# Autodesk Inventor assembly: Elo_sup
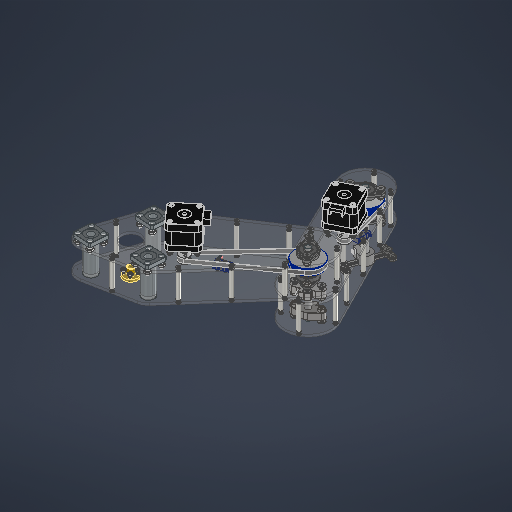
[picture p0: Inventor's stored thumbnail of the model, 512x512]
Saved by Autodesk Inventor 2025.2 (Build 292293000, 293)
## iProperties
Created: 2025-04-19
Part Number: Elo_sup
Document SubType Name: Assembly
Designer: Nelson
Author: Nelson
## Documents named in this file (33)
- C:\Users\Tiago\Documents\Inventor\Exp. Braço v1\Elo_sup.iam
- C:\Users\Tiago\Documents\Inventor\Exp. Braço v1\Veio_D8mm_L100mm.ipt
- C:\Users\Tiago\Documents\Inventor\Exp. Braço v1\RolamentoLinear10d.ipt
- C:\Users\Tiago\Documents\Inventor\Exp. Braço v1\KFL08 - Mancal Flange oval Ø8.ipt
- C:\Users\Tiago\Documents\Inventor\Exp. Braço v1\NEMA17 42-38.ipt
- C:\Users\Tiago\Documents\Inventor\Exp. Braço v1\Porca_T8.ipt
- C:\Users\Tiago\Documents\Inventor\Exp. Braço v1\Linear_Shaft_Support_SHF8.ipt
- C:\Users\Tiago\Documents\Inventor\Exp. Braço v1\1ELO.ipt
- C:\Users\Tiago\Documents\Inventor\Exp. Braço v1\2ELO.ipt
- C:\Users\Tiago\Documents\Inventor\Exp. Braço v1\3ELO.ipt
- C:\Users\Tiago\Documents\Inventor\Exp. Braço v1\4ELO.ipt
- C:\Users\Tiago\Documents\Inventor\Exp. Braço v1\espaçador_M3_L40.ipt
- C:\Users\Tiago\Documents\Inventor\Exp. Braço v1\GT2Pulley_z60.ipt
- C:\Users\Tiago\Documents\Inventor\Exp. Braço v1\GT2Pulley_z20.ipt
- C:\Users\Tiago\Documents\Inventor\Exp. Braço v1\Elo_sup\Design Accelerator\Synchronous Belts Transmission3.iam
- C:\Users\Tiago\Documents\Inventor\Exp. Braço v1\Elo_sup\Design Accelerator\Synchronous Belts Transmission5.iam
- C:\Users\Tiago\Documents\Inventor\Exp. Braço v1\M3 x0.5 ALT (...).ipt
- C:\Users\Tiago\Documents\Inventor\Exp. Braço v1\Anilha_M3.ipt
- C:\Users\Tiago\Documents\Inventor\Exp. Braço v1\M3 x8L_hexagonal_BigHEAD.ipt
- C:\Users\Tiago\Documents\Inventor\Exp. Braço v1\M5x14L_Hex.ipt
- C:\Users\Tiago\Documents\Inventor\Exp. Braço v1\M5_nylonLock_Nut.ipt
- C:\Users\Tiago\Documents\Inventor\Exp. Braço v1\M4x12L_Hex.ipt
- C:\Users\Tiago\Documents\Inventor\Exp. Braço v1\Porca_sextavada(4M).ipt
- C:\Users\Tiago\Documents\Inventor\Exp. Braço v1\M5x16L_Hex.ipt
- C:\Users\Tiago\Documents\Inventor\Exp. Braço v1\M2x12L_Hex.ipt
- M2x12L_Hex.ipt
- C:\Users\Tiago\Documents\Inventor\Exp. Braço v1\Porca_sextavada(M2).ipt
- C:\Users\Tiago\Documents\Inventor\Exp. Braço v1\M5 x12L_Hex_C.ipt
- M5 x12L_Hex_C.ipt
- C:\Users\Tiago\Documents\Inventor\Exp. Braço v1\Porca_sextavada(3M).ipt
- C:\Users\Tiago\Documents\Inventor\Exp. Braço v1\Limit switch\complete limit switch\complete limit switch\complete limit switch.ipt
- C:\Users\Tiago\Documents\Inventor\Exp. Braço v1\EndEffector_holder_Touch.ipt
- C:\Users\Tiago\Documents\Inventor\Exp. Braço v1\EndEffector_Holder_for_SHF.ipt
## Components (176 placed, 29 different names)
1. Veio_D8mm_L100mm:1 — Mate:45, Mate:48, Mate:61, Flush:3, Mate:64, Mate:65, Mate:78, Mate:82, Flush:5, Mate:143, Rotation:3, Rotation:4
2. RolamentoLinear10d:1 — Mate:54, Mate:68, Flush:4, Mate:192, Mate:193, Insert:163, Insert:168, Insert:169, Insert:170
3. RolamentoLinear10d:2 — Mate:56, Mate:190, Mate:191, Insert:159, Insert:160, Insert:161, Insert:162
4. RolamentoLinear10d:3 — Mate:57, Mate:70, Mate:194, Mate:195, Insert:164, Insert:165, Insert:166, Insert:167
5. KFL08 - Mancal Flange oval Ø8:1 — Mate:65, Mate:71, Mate:91, Insert:147, Insert:148
6. KFL08 - Mancal Flange oval Ø8:2 — Mate:63, Mate:64, Mate:74, Mate:75, Insert:149, Insert:150
7. NEMA17 42-38:1 — Mate:98, Mate:141, Mate:144, Flush:161, Mate:201, Mate:202, Mate:203, Mate:204
8. Porca_T8:1 — Mate:66, Mate:67, Mate:76, Mate:77, Insert:199, Insert:200, Insert:201, Insert:202
9. NEMA17 42-38:2 — Mate:162, Mate:163, Mate:164, Flush:159, Mate:197, Mate:198, Mate:199, Mate:200
10. Linear_Shaft_Support_SHF8:1 — Mate:45, Mate:80, Mate:81, Insert:187, Insert:188, Insert:195
11. Linear_Shaft_Support_SHF8:2 — Mate:48, Mate:83, Mate:84, Insert:189, Insert:190, Insert:196
12. Veio_D8mm_L100mm:2 — Mate:51, Mate:53, Mate:85, Mate:86, Flush:6, Mate:149, Flush:162, Mate:211
13. KFL08 - Mancal Flange oval Ø8:3 — Mate:51, Mate:87, Mate:88, Insert:157, Insert:158
14. KFL08 - Mancal Flange oval Ø8:4 — Mate:53, Mate:89, Mate:90, Insert:155, Insert:156
15. 1ELO:1 — Mate:54, Mate:56, Mate:57, Mate:61, Flush:3, Mate:63, Mate:74, Mate:75, Mate:98, Mate:100, Mate:101, Mate:102, Mate:103, Mate:104, Mate:105, Mate:106, Mate:121, Mate:127, Mate:144, Mate:145, Mate:146, Flush:158, Mate:157, Mate:186, Mate:187, Mate:188, Mate:189, Mate:190, Mate:191, Mate:192, Mate:193, Mate:194, Mate:195, Insert:95, Mate:196, Insert:97, Insert:98, Insert:99, Insert:100, Insert:101, Insert:102, Insert:103, Insert:143, Insert:144, Insert:171, Insert:172, Insert:173, Insert:174, Insert:175, Insert:176, Insert:177, Insert:178, Insert:179, Insert:180, Insert:181, Insert:182
16. 2ELO:1 — Mate:66, Mate:67, Mate:68, Mate:70, Flush:4, Mate:71, Mate:76, Mate:77, Distância dos elos, Mate:91, Mate:99, Mate:120, Mate:122, Mate:123, Mate:124, Mate:125, Mate:126, Mate:128, Angle:1, Flush:161, Insert:112, Insert:113, Insert:114, Insert:115, Insert:116, Insert:117, Insert:118, Insert:119, Mate:107, Insert:145, Insert:146, Insert:193, Insert:194, Insert:197, Insert:203, Insert:204, Insert:205, Insert:206, Mate:208, Mate:209, Mate:210
17. 3ELO:1 — Mate:78, Distância dos elos, Mate:80, Mate:81, Mate:85, Flush:6, Mate:87, Mate:88, Mate:129, Mate:130, Mate:131, Mate:132, Mate:133, Mate:134, Mate:135, Mate:136, Mate:137, Mate:138, Mate:139, Mate:140, Rotation:4, Mate:162, Mate:163, Mate:166, Mate:173, Mate:175, Mate:177, Mate:180, Mate:181, Insert:120, Insert:121, Insert:122, Insert:123, Insert:124, Insert:125, Insert:126, Insert:127, Insert:128, Insert:129, Insert:130, Insert:151, Insert:152, Insert:183, Insert:184, Insert:198
18. 4ELO:1 — Mate:82, Flush:5, Mate:83, Mate:84, Mate:86, Mate:89, Mate:90, Mate:108, Mate:109, Mate:110, Mate:111, Mate:112, Mate:113, Mate:114, Mate:115, Mate:116, Mate:117, Mate:118, Mate:119, Angle:1, Mate:167, Flush:159, Mate:173, Insert:131, Insert:132, Insert:133, Insert:134, Insert:135, Insert:136, Insert:137, Insert:138, Insert:139, Insert:140, Insert:141, Insert:142, Insert:153, Insert:154, Insert:185, Insert:186, Mate:205, Mate:206, Mate:207, Angle:2, Insert:217, Insert:218
19. espaçador_M3_L40:1 — Mate:99, Mate:100
20. espaçador_M3_L40:2 — Mate:101, Mate:126
21. espaçador_M3_L40:3 — Mate:103, Mate:123
22. espaçador_M3_L40:4 — Mate:105, Mate:122
23. espaçador_M3_L40:5 — Mate:102, Mate:127
24. espaçador_M3_L40:6 — Mate:107, Mate:125
25. espaçador_M3_L40:7 — Mate:108, Mate:130
26. espaçador_M3_L40:8 — Mate:109, Mate:131
27. espaçador_M3_L40:9 — Mate:104, Mate:128
28. espaçador_M3_L40:10 — Mate:106, Mate:124
29. espaçador_M3_L40:11 — Mate:110, Mate:129
30. espaçador_M3_L40:12 — Mate:111, Mate:135
31. espaçador_M3_L40:13 — Mate:114, Mate:138
32. espaçador_M3_L40:14 — Mate:113, Mate:139
33. espaçador_M3_L40:15 — Mate:112, Mate:140
34. espaçador_M3_L40:16 — Mate:115, Mate:136
35. espaçador_M3_L40:17 — Mate:116, Mate:137
36. espaçador_M3_L40:18 — Mate:117, Mate:134
37. espaçador_M3_L40:20 — Mate:119, Mate:132
38. espaçador_M3_L40:21 — Mate:120, Mate:121
39. espaçador_M3_L40:22 — Mate:118, Mate:133
40. GT2Pulley_z60:1 — Mate:143, Mate:145, Mate:148, Flush:7, Rotation:1, Rotation:3
41. GT2Pulley_z20:1 — Mate:141, Mate:146, Mate:147, Rotation:1
42. Synchronous Belts Transmission:3 [sub-assembly] — Mate:147, Mate:148, Flush:7
43. GT2Pulley_z20:2 — Rotation:2, Mate:164, Mate:167, Mate:169
44. GT2Pulley_z60:2 — Mate:149, Rotation:2, Mate:166, Mate:168, Flush:160
45. Synchronous Belts Transmission:4 [sub-assembly] — Mate:168, Mate:169, Flush:160
46. M3 x0.5 ALT (...):1 — Mate:196
47. M3 x0.5 ALT (...):2 — Insert:95
48. M3 x0.5 ALT (...):3 — Insert:98
49. M3 x0.5 ALT (...):4 — Insert:97
50. M3 x0.5 ALT (...):5 — Insert:99
51. M3 x0.5 ALT (...):6 — Insert:102
52. M3 x0.5 ALT (...):7 — Insert:101
53. M3 x0.5 ALT (...):8 — Insert:100
54. M3 x0.5 ALT (...):9 — Insert:103
55. M3 x0.5 ALT (...):10 — Insert:120
56. M3 x0.5 ALT (...):11 — Insert:198
57. M3 x0.5 ALT (...):12 — Insert:130
58. M3 x0.5 ALT (...):13 — Insert:129
59. M3 x0.5 ALT (...):14 — Insert:116
60. M3 x0.5 ALT (...):15 — Insert:119
61. M3 x0.5 ALT (...):16 — Insert:115
62. M3 x0.5 ALT (...):17 — Insert:121
63. M3 x0.5 ALT (...):18 — Insert:128
64. M3 x0.5 ALT (...):19 — Insert:124
65. M3 x0.5 ALT (...):20 — Insert:126
66. M3 x0.5 ALT (...):21 — Insert:127
67. M3 x0.5 ALT (...):22 — Insert:125
68. M3 x0.5 ALT (...):23 — Insert:122
69. M3 x0.5 ALT (...):24 — Insert:123
70. M3 x0.5 ALT (...):25 — Insert:142
71. M3 x0.5 ALT (...):26 — Insert:141
72. M3 x0.5 ALT (...):27 — Insert:140
73. M3 x0.5 ALT (...):28 — Insert:138
74. M3 x0.5 ALT (...):29 — Insert:139
75. M3 x0.5 ALT (...):30 — Insert:136
76. M3 x0.5 ALT (...):31 — Insert:134
77. M3 x0.5 ALT (...):32 — Insert:137
78. M3 x0.5 ALT (...):33 — Insert:132
79. M3 x0.5 ALT (...):34 — Insert:131
80. M3 x0.5 ALT (...):35 — Insert:133
81. M3 x0.5 ALT (...):36 — Insert:135
82. M3 x0.5 ALT (...):37 — Insert:112
83. M3 x0.5 ALT (...):38 — Insert:197
84. M3 x0.5 ALT (...):39 — Insert:117
85. M3 x0.5 ALT (...):40 — Insert:118
86. M3 x0.5 ALT (...):41 — Insert:114
87. M3 x0.5 ALT (...):42 — Insert:113
88. Anilha_M3:43 — Mate:175, Insert:108
89. Anilha_M3:44 — Mate:177, Insert:109
90. Anilha_M3:45 — Mate:181, Insert:110
91. Anilha_M3:46 — Mate:180, Insert:111
92. Anilha_M3:47 — Mate:187, Insert:104
93. Anilha_M3:48 — Mate:189, Insert:105
94. Anilha_M3:49 — Mate:186, Insert:107
95. Anilha_M3:50 — Mate:188, Insert:106
96. M3 x8L_hexagonal_BigHEAD:1 — Insert:104, Mate:202
97. M3 x8L_hexagonal_BigHEAD:2 — Insert:105, Mate:203
98. M3 x8L_hexagonal_BigHEAD:3 — Insert:107, Mate:201
99. M3 x8L_hexagonal_BigHEAD:4 — Insert:106, Mate:204
100. M3 x8L_hexagonal_BigHEAD:5 — Insert:110, Mate:197
101. M3 x8L_hexagonal_BigHEAD:6 — Insert:111, Mate:198
102. M3 x8L_hexagonal_BigHEAD:7 — Insert:109, Mate:200
103. M3 x8L_hexagonal_BigHEAD:8 — Insert:108, Mate:199
104. M5x14L_Hex:1 — Insert:143
105. M5x14L_Hex:2 — Insert:144
106. M5x14L_Hex:3 — Insert:145
107. M5x14L_Hex:4 — Insert:146
108. M5_nylonLock_Nut:1 — Insert:149
109. M5_nylonLock_Nut:2 — Insert:147
110. M5_nylonLock_Nut:3 — Insert:150
111. M5_nylonLock_Nut:4 — Insert:148
112. M5_nylonLock_Nut:5 — Insert:155
113. M5_nylonLock_Nut:6 — Insert:157
114. M5_nylonLock_Nut:7 — Insert:158
115. M5_nylonLock_Nut:8 — Insert:156
116. M5x14L_Hex:5 — Insert:154
117. M5x14L_Hex:6 — Insert:153
118. M5x14L_Hex:7 — Insert:151
119. M5x14L_Hex:8 — Insert:152
120. M4x12L_Hex:1 — Insert:159
121. M4x12L_Hex:2 — Insert:161
122. M4x12L_Hex:3 — Insert:162
123. M4x12L_Hex:4 — Insert:160
124. M4x12L_Hex:5 — Insert:170
125. M4x12L_Hex:6 — Insert:168
126. M4x12L_Hex:7 — Insert:163
127. M4x12L_Hex:8 — Insert:164
128. M4x12L_Hex:9 — Insert:165
129. M4x12L_Hex:10 — Insert:169
130. M4x12L_Hex:11 — Insert:166
131. M4x12L_Hex:12 — Insert:167
132. Porca_sextavada(4M):1 — Insert:171
133. Porca_sextavada(4M):2 — Insert:174
134. Porca_sextavada(4M):3 — Insert:172
135. Porca_sextavada(4M):4 — Insert:173
136. Porca_sextavada(4M):5 — Insert:178
137. Porca_sextavada(4M):6 — Insert:177
138. Porca_sextavada(4M):7 — Insert:176
139. Porca_sextavada(4M):8 — Insert:175
140. Porca_sextavada(4M):9 — Insert:179
141. Porca_sextavada(4M):10 — Insert:180
142. Porca_sextavada(4M):11 — Insert:181
143. Porca_sextavada(4M):12 — Insert:182
144. M5x16L_Hex:1 — Insert:183
145. M5x16L_Hex:2 — Insert:184
146. M5x16L_Hex:3 — Insert:186
147. M5x16L_Hex:4 — Insert:185
148. M5_nylonLock_Nut:9 — Insert:188
149. M5_nylonLock_Nut:10 — Insert:187
150. M5_nylonLock_Nut:11 — Insert:189
151. M5_nylonLock_Nut:12 — Insert:190
152. M2x12L_Hex:1 — Insert:211
153. M2x12L_Hex:2 — Insert:210
154. Porca_sextavada(M2):1 — Insert:194
155. Porca_sextavada(M2):2 — Insert:193
156. M5 x12L_Hex_C:1 — Insert:195
157. M5 x12L_Hex_C:2 — Insert:196
158. M3 x0.5 ALT (...):43 — Insert:201
159. M3 x0.5 ALT (...):44 — Insert:202
160. M3 x0.5 ALT (...):45 — Insert:199
161. M3 x0.5 ALT (...):46 — Insert:200
162. Porca_sextavada(3M):1 — Insert:203
163. Porca_sextavada(3M):2 — Insert:206
164. Porca_sextavada(3M):3 — Insert:205
165. Porca_sextavada(3M):4 — Insert:204
166. complete limit switch:1 — Mate:205, Mate:206, Mate:207, Insert:215, Insert:216
167. espaçador_M3_L40:23 — Insert:209, Insert:214
168. M3 x0.5 ALT (...):47 — Insert:213
169. EndEffector_holder_Touch:1 — Insert:209
170. complete limit switch:2 — Mate:208, Mate:209, Mate:210, Insert:210, Insert:211
171. EndEffector_Holder_for_SHF:1 — Flush:162, Mate:211, Insert:212, Insert:213, Insert:214, Angle:2
172. M5 x12L_Hex_C:3 — Insert:212
173. M2x12L_Hex:3 — Insert:216
174. M2x12L_Hex:4 — Insert:215
175. Porca_sextavada(M2):3 — Insert:217
176. Porca_sextavada(M2):4 — Insert:218
## Relationships (260: Mate 124, Insert 119, Flush 11, RelateRotation 4, Angle 2)
- Flush:2 (-10 mm)
- Mate:45: Veio_D8mm_L100mm:1 ↔ Linear_Shaft_Support_SHF8:1
- Mate:48: Veio_D8mm_L100mm:1 ↔ Linear_Shaft_Support_SHF8:2
- Mate:51: Veio_D8mm_L100mm:2 ↔ KFL08 - Mancal Flange oval Ø8:3
- Mate:53: Veio_D8mm_L100mm:2 ↔ KFL08 - Mancal Flange oval Ø8:4
- Mate:54: RolamentoLinear10d:1 ↔ 1ELO:1
- Mate:56: RolamentoLinear10d:2 ↔ 1ELO:1
- Mate:57: RolamentoLinear10d:3 ↔ 1ELO:1
- Mate:61: Veio_D8mm_L100mm:1 ↔ 1ELO:1
- Flush:3 (-1 mm): Veio_D8mm_L100mm:1 ↔ 1ELO:1
- Mate:63: KFL08 - Mancal Flange oval Ø8:2 ↔ 1ELO:1
- Mate:64: Veio_D8mm_L100mm:1 ↔ KFL08 - Mancal Flange oval Ø8:2
- Mate:65: Veio_D8mm_L100mm:1 ↔ KFL08 - Mancal Flange oval Ø8:1
- Mate:66: Porca_T8:1 ↔ 2ELO:1
- Mate:67: Porca_T8:1 ↔ 2ELO:1
- Mate:68: RolamentoLinear10d:1 ↔ 2ELO:1
- Mate:70: RolamentoLinear10d:3 ↔ 2ELO:1
- Flush:4 (-1 mm): RolamentoLinear10d:1 ↔ 2ELO:1
- Mate:71: KFL08 - Mancal Flange oval Ø8:1 ↔ 2ELO:1
- Mate:74: KFL08 - Mancal Flange oval Ø8:2 ↔ 1ELO:1
- Mate:75: KFL08 - Mancal Flange oval Ø8:2 ↔ 1ELO:1
- Mate:76: Porca_T8:1 ↔ 2ELO:1
- Mate:77: Porca_T8:1 ↔ 2ELO:1
- Mate:78: Veio_D8mm_L100mm:1 ↔ 3ELO:1
- Distância dos elos [Mate] (3 mm): 2ELO:1 ↔ 3ELO:1
- Mate:80: Linear_Shaft_Support_SHF8:1 ↔ 3ELO:1
- Mate:81: Linear_Shaft_Support_SHF8:1 ↔ 3ELO:1
- Mate:82: Veio_D8mm_L100mm:1 ↔ 4ELO:1
- Flush:5: Veio_D8mm_L100mm:1 ↔ 4ELO:1
- Mate:83: Linear_Shaft_Support_SHF8:2 ↔ 4ELO:1
- Mate:84: Linear_Shaft_Support_SHF8:2 ↔ 4ELO:1
- Mate:85: Veio_D8mm_L100mm:2 ↔ 3ELO:1
- Mate:86: Veio_D8mm_L100mm:2 ↔ 4ELO:1
- Flush:6: Veio_D8mm_L100mm:2 ↔ 3ELO:1
- Mate:87: KFL08 - Mancal Flange oval Ø8:3 ↔ 3ELO:1
- Mate:88: KFL08 - Mancal Flange oval Ø8:3 ↔ 3ELO:1
- Mate:89: KFL08 - Mancal Flange oval Ø8:4 ↔ 4ELO:1
- Mate:90: KFL08 - Mancal Flange oval Ø8:4 ↔ 4ELO:1
- Mate:91: KFL08 - Mancal Flange oval Ø8:1 ↔ 2ELO:1
- Mate:98: NEMA17 42-38:1 ↔ 1ELO:1
- Mate:99: 2ELO:1 ↔ espaçador_M3_L40:1
- Mate:100: 1ELO:1 ↔ espaçador_M3_L40:1
- Mate:101: 1ELO:1 ↔ espaçador_M3_L40:2
- Mate:102: 1ELO:1 ↔ espaçador_M3_L40:5
- Mate:103: 1ELO:1 ↔ espaçador_M3_L40:3
- Mate:104: 1ELO:1 ↔ espaçador_M3_L40:9
- Mate:105: 1ELO:1 ↔ espaçador_M3_L40:4
- Mate:106: 1ELO:1 ↔ espaçador_M3_L40:10
- Mate:107: 2ELO:1 ↔ espaçador_M3_L40:6
- Mate:108: 4ELO:1 ↔ espaçador_M3_L40:7
- Mate:109: 4ELO:1 ↔ espaçador_M3_L40:8
- Mate:110: 4ELO:1 ↔ espaçador_M3_L40:11
- Mate:111: 4ELO:1 ↔ espaçador_M3_L40:12
- Mate:112: 4ELO:1 ↔ espaçador_M3_L40:15
- Mate:113: 4ELO:1 ↔ espaçador_M3_L40:14
- Mate:114: 4ELO:1 ↔ espaçador_M3_L40:13
- Mate:115: 4ELO:1 ↔ espaçador_M3_L40:16
- Mate:116: 4ELO:1 ↔ espaçador_M3_L40:17
- Mate:117: 4ELO:1 ↔ espaçador_M3_L40:18
- Mate:118: 4ELO:1 ↔ espaçador_M3_L40:22
- Mate:119: 4ELO:1 ↔ espaçador_M3_L40:20
- Mate:120: 2ELO:1 ↔ espaçador_M3_L40:21
- Mate:121: 1ELO:1 ↔ espaçador_M3_L40:21
- Mate:122: 2ELO:1 ↔ espaçador_M3_L40:4
- Mate:123: 2ELO:1 ↔ espaçador_M3_L40:3
- Mate:124: 2ELO:1 ↔ espaçador_M3_L40:10
- Mate:125: 2ELO:1 ↔ espaçador_M3_L40:6
- Mate:126: 2ELO:1 ↔ espaçador_M3_L40:2
- Mate:127: 1ELO:1 ↔ espaçador_M3_L40:5
- Mate:128: 2ELO:1 ↔ espaçador_M3_L40:9
- Mate:129: 3ELO:1 ↔ espaçador_M3_L40:11
- Mate:130: 3ELO:1 ↔ espaçador_M3_L40:7
- Mate:131: 3ELO:1 ↔ espaçador_M3_L40:8
- Mate:132: 3ELO:1 ↔ espaçador_M3_L40:20
- Mate:133: 3ELO:1 ↔ espaçador_M3_L40:22
- Mate:134: 3ELO:1 ↔ espaçador_M3_L40:18
- Mate:135: 3ELO:1 ↔ espaçador_M3_L40:12
- Mate:136: 3ELO:1 ↔ espaçador_M3_L40:16
- Mate:137: 3ELO:1 ↔ espaçador_M3_L40:17
- Mate:138: 3ELO:1 ↔ espaçador_M3_L40:13
- Mate:139: 3ELO:1 ↔ espaçador_M3_L40:14
- Mate:140: 3ELO:1 ↔ espaçador_M3_L40:15
- Mate:141: NEMA17 42-38:1 ↔ GT2Pulley_z20:1
- Mate:143: Veio_D8mm_L100mm:1 ↔ GT2Pulley_z60:1
- Mate:144: NEMA17 42-38:1 ↔ 1ELO:1
- Mate:145 (12 mm): 1ELO:1 ↔ GT2Pulley_z60:1
- Mate:146 (6.6 mm): 1ELO:1 ↔ GT2Pulley_z20:1
- Mate:147: GT2Pulley_z20:1 ↔ Synchronous Belts Transmission:3
- Mate:148: GT2Pulley_z60:1 ↔ Synchronous Belts Transmission:3
- Flush:7 (2.5 mm): GT2Pulley_z60:1 ↔ Synchronous Belts Transmission:3
- Rotation:1 [RelateRotation] (3 ul): GT2Pulley_z60:1 ↔ GT2Pulley_z20:1
- Mate:149: Veio_D8mm_L100mm:2 ↔ GT2Pulley_z60:2
- Rotation:2 [RelateRotation] (3 ul): GT2Pulley_z20:2 ↔ GT2Pulley_z60:2
- Flush:158: 1ELO:1
- Mate:157: 1ELO:1
- Rotation:3 [RelateRotation] (1 ul): Veio_D8mm_L100mm:1 ↔ GT2Pulley_z60:1
- Rotation:4 [RelateRotation] (1 ul): Veio_D8mm_L100mm:1 ↔ 3ELO:1
- Angle:1 (135 deg): 2ELO:1 ↔ 4ELO:1
- Mate:162: NEMA17 42-38:2 ↔ 3ELO:1
- Mate:163: NEMA17 42-38:2 ↔ 3ELO:1
- Mate:164: NEMA17 42-38:2 ↔ GT2Pulley_z20:2
- Mate:166 (12 mm): 3ELO:1 ↔ GT2Pulley_z60:2
- Mate:167 (17.6 mm): 4ELO:1 ↔ GT2Pulley_z20:2
- Flush:159 (141.105 mm): NEMA17 42-38:2 ↔ 4ELO:1
- Mate:168: GT2Pulley_z60:2 ↔ Synchronous Belts Transmission:4
- Mate:169: GT2Pulley_z20:2 ↔ Synchronous Belts Transmission:4
- Flush:160 (-2.2 mm): GT2Pulley_z60:2 ↔ Synchronous Belts Transmission:4
- Mate:173 (40 mm): 3ELO:1 ↔ 4ELO:1
- Flush:161 (99.63 mm): NEMA17 42-38:1 ↔ 2ELO:1
- Mate:175: 3ELO:1 ↔ Anilha_M3:43
- Mate:177: 3ELO:1 ↔ Anilha_M3:44
- Mate:180: 3ELO:1 ↔ Anilha_M3:46
- Mate:181: 3ELO:1 ↔ Anilha_M3:45
- Mate:186: 1ELO:1 ↔ Anilha_M3:49
- Mate:187: 1ELO:1 ↔ Anilha_M3:47
- Mate:188: 1ELO:1 ↔ Anilha_M3:50
- Mate:189: 1ELO:1 ↔ Anilha_M3:48
- Mate:190: RolamentoLinear10d:2 ↔ 1ELO:1
- Mate:191: RolamentoLinear10d:2 ↔ 1ELO:1
- Mate:192: RolamentoLinear10d:1 ↔ 1ELO:1
- Mate:193: RolamentoLinear10d:1 ↔ 1ELO:1
- Mate:194: RolamentoLinear10d:3 ↔ 1ELO:1
- Mate:195: RolamentoLinear10d:3 ↔ 1ELO:1
- Insert:95: 1ELO:1 ↔ M3 x0.5 ALT (...):2
- Mate:196: 1ELO:1 ↔ M3 x0.5 ALT (...):1
- Insert:97: 1ELO:1 ↔ M3 x0.5 ALT (...):4
- Insert:98: 1ELO:1 ↔ M3 x0.5 ALT (...):3
- Insert:99: 1ELO:1 ↔ M3 x0.5 ALT (...):5
- Insert:100: 1ELO:1 ↔ M3 x0.5 ALT (...):8
- Insert:101: 1ELO:1 ↔ M3 x0.5 ALT (...):7
- Insert:102: 1ELO:1 ↔ M3 x0.5 ALT (...):6
- Insert:103: 1ELO:1 ↔ M3 x0.5 ALT (...):9
- Insert:104: Anilha_M3:47 ↔ M3 x8L_hexagonal_BigHEAD:1
- Insert:105: Anilha_M3:48 ↔ M3 x8L_hexagonal_BigHEAD:2
- Insert:106: Anilha_M3:50 ↔ M3 x8L_hexagonal_BigHEAD:4
- Insert:107: Anilha_M3:49 ↔ M3 x8L_hexagonal_BigHEAD:3
- Insert:108: Anilha_M3:43 ↔ M3 x8L_hexagonal_BigHEAD:8
- Insert:109: Anilha_M3:44 ↔ M3 x8L_hexagonal_BigHEAD:7
- Insert:110: Anilha_M3:45 ↔ M3 x8L_hexagonal_BigHEAD:5
- Insert:111: Anilha_M3:46 ↔ M3 x8L_hexagonal_BigHEAD:6
- Insert:112: 2ELO:1 ↔ M3 x0.5 ALT (...):37
- Insert:113: 2ELO:1 ↔ M3 x0.5 ALT (...):42
- Insert:114: 2ELO:1 ↔ M3 x0.5 ALT (...):41
- Insert:115: 2ELO:1 ↔ M3 x0.5 ALT (...):16
- Insert:116: 2ELO:1 ↔ M3 x0.5 ALT (...):14
- Insert:117: 2ELO:1 ↔ M3 x0.5 ALT (...):39
- Insert:118: 2ELO:1 ↔ M3 x0.5 ALT (...):40
- Insert:119: 2ELO:1 ↔ M3 x0.5 ALT (...):15
- Insert:120: 3ELO:1 ↔ M3 x0.5 ALT (...):10
- Insert:121: 3ELO:1 ↔ M3 x0.5 ALT (...):17
- Insert:122: 3ELO:1 ↔ M3 x0.5 ALT (...):23
- Insert:123: 3ELO:1 ↔ M3 x0.5 ALT (...):24
- Insert:124: 3ELO:1 ↔ M3 x0.5 ALT (...):19
- Insert:125: 3ELO:1 ↔ M3 x0.5 ALT (...):22
- Insert:126: 3ELO:1 ↔ M3 x0.5 ALT (...):20
- Insert:127: 3ELO:1 ↔ M3 x0.5 ALT (...):21
- Insert:128: 3ELO:1 ↔ M3 x0.5 ALT (...):18
- Insert:129: 3ELO:1 ↔ M3 x0.5 ALT (...):13
- Insert:130: 3ELO:1 ↔ M3 x0.5 ALT (...):12
- Insert:131: 4ELO:1 ↔ M3 x0.5 ALT (...):34
- Insert:132: 4ELO:1 ↔ M3 x0.5 ALT (...):33
- Insert:133: 4ELO:1 ↔ M3 x0.5 ALT (...):35
- Insert:134: 4ELO:1 ↔ M3 x0.5 ALT (...):31
- Insert:135: 4ELO:1 ↔ M3 x0.5 ALT (...):36
- Insert:136: 4ELO:1 ↔ M3 x0.5 ALT (...):30
- Insert:137: 4ELO:1 ↔ M3 x0.5 ALT (...):32
- Insert:138: 4ELO:1 ↔ M3 x0.5 ALT (...):28
- Insert:139: 4ELO:1 ↔ M3 x0.5 ALT (...):29
- Insert:140: 4ELO:1 ↔ M3 x0.5 ALT (...):27
- Insert:141: 4ELO:1 ↔ M3 x0.5 ALT (...):26
- Insert:142: 4ELO:1 ↔ M3 x0.5 ALT (...):25
- Mate:197: NEMA17 42-38:2 ↔ M3 x8L_hexagonal_BigHEAD:5
- Mate:198: NEMA17 42-38:2 ↔ M3 x8L_hexagonal_BigHEAD:6
- Mate:199: NEMA17 42-38:2 ↔ M3 x8L_hexagonal_BigHEAD:8
- Mate:200: NEMA17 42-38:2 ↔ M3 x8L_hexagonal_BigHEAD:7
- Mate:201: NEMA17 42-38:1 ↔ M3 x8L_hexagonal_BigHEAD:3
- Mate:202: NEMA17 42-38:1 ↔ M3 x8L_hexagonal_BigHEAD:1
- Mate:203: NEMA17 42-38:1 ↔ M3 x8L_hexagonal_BigHEAD:2
- Mate:204: NEMA17 42-38:1 ↔ M3 x8L_hexagonal_BigHEAD:4
- Insert:143: 1ELO:1 ↔ M5x14L_Hex:1
- Insert:144: 1ELO:1 ↔ M5x14L_Hex:2
- Insert:145: 2ELO:1 ↔ M5x14L_Hex:3
- Insert:146: 2ELO:1 ↔ M5x14L_Hex:4
- Insert:147: KFL08 - Mancal Flange oval Ø8:1 ↔ M5_nylonLock_Nut:2
- Insert:148: KFL08 - Mancal Flange oval Ø8:1 ↔ M5_nylonLock_Nut:4
- Insert:149: KFL08 - Mancal Flange oval Ø8:2 ↔ M5_nylonLock_Nut:1
- Insert:150: KFL08 - Mancal Flange oval Ø8:2 ↔ M5_nylonLock_Nut:3
- Insert:151: 3ELO:1 ↔ M5x14L_Hex:7
- Insert:152: 3ELO:1 ↔ M5x14L_Hex:8
- Insert:153: 4ELO:1 ↔ M5x14L_Hex:6
- Insert:154: 4ELO:1 ↔ M5x14L_Hex:5
- Insert:155: KFL08 - Mancal Flange oval Ø8:4 ↔ M5_nylonLock_Nut:5
- Insert:156: KFL08 - Mancal Flange oval Ø8:4 ↔ M5_nylonLock_Nut:8
- Insert:157: KFL08 - Mancal Flange oval Ø8:3 ↔ M5_nylonLock_Nut:6
- Insert:158: KFL08 - Mancal Flange oval Ø8:3 ↔ M5_nylonLock_Nut:7
- Insert:159: RolamentoLinear10d:2 ↔ M4x12L_Hex:1
- Insert:160: RolamentoLinear10d:2 ↔ M4x12L_Hex:4
- Insert:161: RolamentoLinear10d:2 ↔ M4x12L_Hex:2
- Insert:162: RolamentoLinear10d:2 ↔ M4x12L_Hex:3
- Insert:163: RolamentoLinear10d:1 ↔ M4x12L_Hex:7
- Insert:164: RolamentoLinear10d:3 ↔ M4x12L_Hex:8
- Insert:165: RolamentoLinear10d:3 ↔ M4x12L_Hex:9
- Insert:166: RolamentoLinear10d:3 ↔ M4x12L_Hex:11
- Insert:167: RolamentoLinear10d:3 ↔ M4x12L_Hex:12
- Insert:168: RolamentoLinear10d:1 ↔ M4x12L_Hex:6
- Insert:169: RolamentoLinear10d:1 ↔ M4x12L_Hex:10
- Insert:170: RolamentoLinear10d:1 ↔ M4x12L_Hex:5
- Insert:171: 1ELO:1 ↔ Porca_sextavada(4M):1
- Insert:172: 1ELO:1 ↔ Porca_sextavada(4M):3
- Insert:173: 1ELO:1 ↔ Porca_sextavada(4M):4
- Insert:174: 1ELO:1 ↔ Porca_sextavada(4M):2
- Insert:175: 1ELO:1 ↔ Porca_sextavada(4M):8
- Insert:176: 1ELO:1 ↔ Porca_sextavada(4M):7
- Insert:177: 1ELO:1 ↔ Porca_sextavada(4M):6
- Insert:178: 1ELO:1 ↔ Porca_sextavada(4M):5
- Insert:179: 1ELO:1 ↔ Porca_sextavada(4M):9
- Insert:180: 1ELO:1 ↔ Porca_sextavada(4M):10
- Insert:181: 1ELO:1 ↔ Porca_sextavada(4M):11
- Insert:182: 1ELO:1 ↔ Porca_sextavada(4M):12
- Insert:183: 3ELO:1 ↔ M5x16L_Hex:1
- Insert:184: 3ELO:1 ↔ M5x16L_Hex:2
- Insert:185: 4ELO:1 ↔ M5x16L_Hex:4
- Insert:186: 4ELO:1 ↔ M5x16L_Hex:3
- Insert:187: Linear_Shaft_Support_SHF8:1 ↔ M5_nylonLock_Nut:10
- Insert:188: Linear_Shaft_Support_SHF8:1 ↔ M5_nylonLock_Nut:9
- Insert:189: Linear_Shaft_Support_SHF8:2 ↔ M5_nylonLock_Nut:11
- Insert:190: Linear_Shaft_Support_SHF8:2 ↔ M5_nylonLock_Nut:12
- Insert:193: 2ELO:1 ↔ Porca_sextavada(M2):2
- Insert:194: 2ELO:1 ↔ Porca_sextavada(M2):1
- Insert:195: Linear_Shaft_Support_SHF8:1 ↔ M5 x12L_Hex_C:1
- Insert:196: Linear_Shaft_Support_SHF8:2 ↔ M5 x12L_Hex_C:2
- Insert:197: 2ELO:1 ↔ M3 x0.5 ALT (...):38
- Insert:198: 3ELO:1 ↔ M3 x0.5 ALT (...):11
- Insert:199: Porca_T8:1 ↔ M3 x0.5 ALT (...):45
- Insert:200: Porca_T8:1 ↔ M3 x0.5 ALT (...):46
- Insert:201: Porca_T8:1 ↔ M3 x0.5 ALT (...):43
- Insert:202: Porca_T8:1 ↔ M3 x0.5 ALT (...):44
- Insert:203: 2ELO:1 ↔ Porca_sextavada(3M):1
- Insert:204: 2ELO:1 ↔ Porca_sextavada(3M):4
- Insert:205: 2ELO:1 ↔ Porca_sextavada(3M):3
- Insert:206: 2ELO:1 ↔ Porca_sextavada(3M):2
- Mate:205: 4ELO:1 ↔ complete limit switch:1
- Mate:206: 4ELO:1 ↔ complete limit switch:1
- Mate:207: 4ELO:1 ↔ complete limit switch:1
- Insert:209: espaçador_M3_L40:23 ↔ EndEffector_holder_Touch:1
- Mate:208: 2ELO:1 ↔ complete limit switch:2
- Mate:209: 2ELO:1 ↔ complete limit switch:2
- Mate:210: 2ELO:1 ↔ complete limit switch:2
- Insert:210: M2x12L_Hex:2 ↔ complete limit switch:2
- Insert:211: M2x12L_Hex:1 ↔ complete limit switch:2
- Flush:162: Veio_D8mm_L100mm:2 ↔ EndEffector_Holder_for_SHF:1
- Mate:211: Veio_D8mm_L100mm:2 ↔ EndEffector_Holder_for_SHF:1
- Insert:212: EndEffector_Holder_for_SHF:1 ↔ M5 x12L_Hex_C:3
- Insert:213: M3 x0.5 ALT (...):47 ↔ EndEffector_Holder_for_SHF:1
- Insert:214: espaçador_M3_L40:23 ↔ EndEffector_Holder_for_SHF:1
- Angle:2 (135 deg): 4ELO:1 ↔ EndEffector_Holder_for_SHF:1
- Insert:215: complete limit switch:1 ↔ M2x12L_Hex:4
- Insert:216: complete limit switch:1 ↔ M2x12L_Hex:3
- Insert:217: 4ELO:1 ↔ Porca_sextavada(M2):3
- Insert:218: 4ELO:1 ↔ Porca_sextavada(M2):4
